# Autodesk Inventor assembly: 3DModel_2
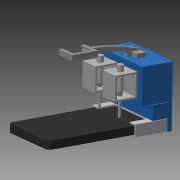
[picture p0: Inventor's stored thumbnail of the model, 180x180]
Saved by Autodesk Inventor 2015 (Build 190159000, 159)
## iProperties
Created: 2015-11-10
Part Number: 3DModel_2
Document SubType Name: Assembly
Designer: Lauszus
Author: Lauszus
## Documents named in this file (8)
- C:\Users\Lauszus\Dropbox\DTU\7. semester\Image Analysis with Microcomputer - 30330\LabExercises\ZomBuster\3DModel\3DModel.iam
- C:\Users\Lauszus\Dropbox\DTU\7. semester\Image Analysis with Microcomputer - 30330\LabExercises\ZomBuster\3DModel\PhoneHolder.ipt
- C:\Users\Lauszus\Dropbox\DTU\7. semester\Image Analysis with Microcomputer - 30330\LabExercises\ZomBuster\3DModel\Solenoid.iam
- C:\Users\Lauszus\Dropbox\DTU\7. semester\Image Analysis with Microcomputer - 30330\LabExercises\ZomBuster\3DModel\Nexus4.ipt
- C:\Users\Lauszus\Dropbox\DTU\7. semester\Image Analysis with Microcomputer - 30330\LabExercises\ZomBuster\3DModel\MachineScrew3mm.ipt
- C:\Users\Lauszus\Dropbox\DTU\7. semester\Image Analysis with Microcomputer - 30330\LabExercises\ZomBuster\3DModel\Back_plate.ipt
- C:\Users\Lauszus\Dropbox\DTU\7. semester\Image Analysis with Microcomputer - 30330\LabExercises\ZomBuster\3DModel\Solenoids_holder.ipt
- C:\Users\Lauszus\Dropbox\DTU\7. semester\Image Analysis with Microcomputer - 30330\LabExercises\ZomBuster\3DModel\CameraAssembly.iam
## Components (11 placed, 7 different names)
1. PhoneHolder:1 — Mate:9, Mate:11, Mate:12, Flush:1, Flush:2, Mate:19, Flush:5, Mate:24, Mate:25
2. Nexus4:1 — Mate:11, Mate:12, Mate:25
3. Back_plate:1 — Flush:1, Flush:2, Flush:3, Flush:4, Mate:18, Mate:24
4. Solenoids_holder:1 — Flush:3, Flush:4, Mate:18, Mate:20, Mate:21, Mate:22, Mate:23, Transitional:1, Transitional:2, Transitional:3, Transitional:4, Mate:26, Flush:7, Flush:8
5. MachineScrew3mm:1 — Mate:20, Transitional:1, Insert:1
6. MachineScrew3mm:2 — Mate:21, Transitional:2, Insert:2
7. MachineScrew3mm:3 — Mate:22, Transitional:3, Insert:3
8. MachineScrew3mm:4 — Mate:23, Transitional:4, Insert:4
9. Solenoid:1 [sub-assembly] — Flush:6, Insert:1, Insert:2
10. Solenoid:2 [sub-assembly] — Flush:6, Insert:3, Insert:4
11. CameraAssembly:1 [sub-assembly] — Mate:26, Flush:7, Flush:8
## Relationships (28: Mate 12, Flush 8, Transitional 4, Insert 4)
- Mate:9: PhoneHolder:1
- Mate:11: PhoneHolder:1 ↔ Nexus4:1
- Mate:12: PhoneHolder:1 ↔ Nexus4:1
- Flush:1: PhoneHolder:1 ↔ Back_plate:1
- Flush:2: PhoneHolder:1 ↔ Back_plate:1
- Flush:3: Back_plate:1 ↔ Solenoids_holder:1
- Flush:4: Back_plate:1 ↔ Solenoids_holder:1
- Mate:18: Back_plate:1 ↔ Solenoids_holder:1
- Mate:19: PhoneHolder:1
- Flush:5: PhoneHolder:1
- Flush:6: Solenoid:1 ↔ Solenoid:2
- Mate:20: Solenoids_holder:1 ↔ MachineScrew3mm:1
- Mate:21: Solenoids_holder:1 ↔ MachineScrew3mm:2
- Mate:22: Solenoids_holder:1 ↔ MachineScrew3mm:3
- Mate:23: Solenoids_holder:1 ↔ MachineScrew3mm:4
- Transitional:1: Solenoids_holder:1 ↔ MachineScrew3mm:1
- Transitional:2: Solenoids_holder:1 ↔ MachineScrew3mm:2
- Transitional:3: Solenoids_holder:1 ↔ MachineScrew3mm:3
- Transitional:4: Solenoids_holder:1 ↔ MachineScrew3mm:4
- Insert:1: MachineScrew3mm:1 ↔ Solenoid:1
- Insert:2: MachineScrew3mm:2 ↔ Solenoid:1
- Insert:3: MachineScrew3mm:3 ↔ Solenoid:2
- Insert:4: MachineScrew3mm:4 ↔ Solenoid:2
- Mate:24: PhoneHolder:1 ↔ Back_plate:1
- Mate:25: PhoneHolder:1 ↔ Nexus4:1
- Mate:26: Solenoids_holder:1 ↔ CameraAssembly:1
- Flush:7 (-5 mm): Solenoids_holder:1 ↔ CameraAssembly:1
- Flush:8 (23.9 mm): Solenoids_holder:1 ↔ CameraAssembly:1
